# Autodesk Inventor assembly: EnsamblajeDodecaedro_V3
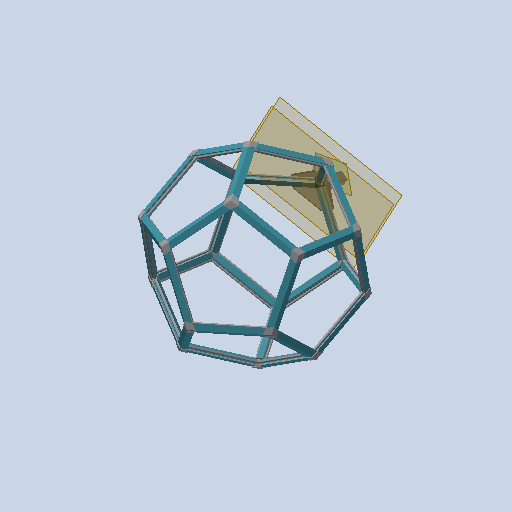
[picture p0: Inventor's stored thumbnail of the model, 512x512]
Saved by Autodesk Inventor 2024 (Build 280153000, 153)
## iProperties
Created: 2023-08-17
Part Number: EnsamblajeDodecaedro_V3
Document SubType Name: Assembly
Designer: sergi
Author: sergi
## Documents named in this file (5)
- C:\Users\sergi\OneDrive\Escritorio\Projects\01. Infinity dodecahedron\Inventor\EnsamblajeDodecaedro_V3.iam
- C:\Users\sergi\OneDrive\Escritorio\Projects\01. Infinity dodecahedron\Inventor\Perfil_V3.ipt
- C:\Users\sergi\OneDrive\Escritorio\Projects\01. Infinity dodecahedron\Inventor\Union.ipt
- C:\Users\sergi\OneDrive\Escritorio\Projects\01. Infinity dodecahedron\Inventor\UnionEntrada.ipt
- C:\Users\sergi\OneDrive\Escritorio\Projects\01. Infinity dodecahedron\Inventor\Base.ipt
## Components (51 placed, 4 different names)
1. Perfil_V3:4 — Coincidencia:1, Coincidencia:2, Coincidencia:3, Coincidencia:19, Coincidencia:20, Coincidencia:21, Coincidencia:154, Coincidencia:155
2. Perfil_V3:5 — Coincidencia:4, Coincidencia:5, Coincidencia:6, Coincidencia:10, Coincidencia:11, Coincidencia:12, Coincidencia:156
3. Perfil_V3:16 — Coincidencia:28, Coincidencia:29, Coincidencia:30, Coincidencia:31, Coincidencia:32, Coincidencia:33
4. Perfil_V3:18 — Coincidencia:7, Coincidencia:8, Coincidencia:9, Coincidencia:55, Coincidencia:56, Coincidencia:57
5. Perfil_V3:25 — Coincidencia:13, Coincidencia:14, Coincidencia:15, Coincidencia:37, Coincidencia:38, Coincidencia:39
6. Perfil_V3:26 — Coincidencia:22, Coincidencia:23, Coincidencia:24, Coincidencia:25, Coincidencia:26, Coincidencia:27
7. Perfil_V3:30 — Coincidencia:16, Coincidencia:17, Coincidencia:18
8. Union:5 — Coincidencia:10, Coincidencia:11, Coincidencia:12, Coincidencia:13, Coincidencia:14, Coincidencia:15, Coincidencia:16, Coincidencia:17, Coincidencia:18
9. Union:6 — Coincidencia:19, Coincidencia:20, Coincidencia:21, Coincidencia:22, Coincidencia:23, Coincidencia:24, Coincidencia:64, Coincidencia:65, Coincidencia:66
10. UnionEntrada:1 — Coincidencia:1, Coincidencia:2, Coincidencia:3, Coincidencia:4, Coincidencia:5, Coincidencia:6, Coincidencia:7, Coincidencia:8, Coincidencia:9
11. Union:7 — Coincidencia:25, Coincidencia:26, Coincidencia:27, Coincidencia:28, Coincidencia:29, Coincidencia:30, Coincidencia:73, Coincidencia:74, Coincidencia:75
12. Union:8 — Coincidencia:31, Coincidencia:32, Coincidencia:33, Coincidencia:34, Coincidencia:35, Coincidencia:36
13. Union:9 — Coincidencia:37, Coincidencia:38, Coincidencia:39, Coincidencia:46, Coincidencia:47, Coincidencia:48, Coincidencia:76, Coincidencia:77, Coincidencia:78
14. Perfil_V3:31 — Coincidencia:34, Coincidencia:35, Coincidencia:36, Coincidencia:79, Coincidencia:80, Coincidencia:81
15. Perfil_V3:32 — Coincidencia:124, Coincidencia:125, Coincidencia:126
16. Perfil_V3:33 — Coincidencia:46, Coincidencia:47, Coincidencia:48
17. Union:10
18. Perfil_V3:34
19. Perfil_V3:35
20. Union:11 — Coincidencia:55, Coincidencia:56, Coincidencia:57
21. Perfil_V3:36
22. Perfil_V3:37 — Coincidencia:64, Coincidencia:65, Coincidencia:66
23. Union:12
24. Perfil_V3:38 — Coincidencia:76, Coincidencia:77, Coincidencia:78
25. Perfil_V3:39 — Coincidencia:73, Coincidencia:74, Coincidencia:75, Coincidencia:106, Coincidencia:107, Coincidencia:114
26. Union:13 — Coincidencia:121, Coincidencia:122, Coincidencia:123
27. Perfil_V3:40
28. Union:14 — Coincidencia:79, Coincidencia:80, Coincidencia:81
29. Perfil_V3:41
30. Perfil_V3:42 — Coincidencia:143
31. Union:15 — Coincidencia:106, Coincidencia:107, Coincidencia:114
32. Union:17 — Coincidencia:148, Coincidencia:149, Coincidencia:150
33. Perfil_V3:44
34. Union:18
35. Perfil_V3:45 — Coincidencia:111, Coincidencia:112, Coincidencia:113
36. Union:19 — Coincidencia:111, Coincidencia:112, Coincidencia:113
37. Perfil_V3:46 — Coincidencia:142, Coincidencia:144
38. Perfil_V3:47 — Coincidencia:121, Coincidencia:122, Coincidencia:123
39. Union:20 — Coincidencia:151, Coincidencia:152, Coincidencia:153
40. Perfil_V3:48
41. Union:21 — Coincidencia:124, Coincidencia:125, Coincidencia:126, Coincidencia:133, Coincidencia:134, Coincidencia:135
42. Perfil_V3:49 — Coincidencia:133, Coincidencia:134, Coincidencia:135
43. Union:22 — Coincidencia:139, Coincidencia:140, Coincidencia:141
44. Perfil_V3:50
45. Union:23 — Coincidencia:142, Coincidencia:143, Coincidencia:144, Coincidencia:145, Coincidencia:146, Coincidencia:147
46. Union:24
47. Perfil_V3:51 — Coincidencia:139, Coincidencia:140, Coincidencia:141
48. Perfil_V3:52 — Coincidencia:145, Coincidencia:146, Coincidencia:147
49. Perfil_V3:53 — Coincidencia:148, Coincidencia:149, Coincidencia:150
50. Perfil_V3:54 — Coincidencia:151, Coincidencia:152, Coincidencia:153
51. Base:1 — Coincidencia:154, Coincidencia:155, Coincidencia:156
## Relationships (150: Mate 150)
- Coincidencia:1 [Mate]: Perfil_V3:4 ↔ UnionEntrada:1
- Coincidencia:2 [Mate]: Perfil_V3:4 ↔ UnionEntrada:1
- Coincidencia:3 [Mate]: Perfil_V3:4 ↔ UnionEntrada:1
- Coincidencia:4 [Mate]: Perfil_V3:5 ↔ UnionEntrada:1
- Coincidencia:5 [Mate]: Perfil_V3:5 ↔ UnionEntrada:1
- Coincidencia:6 [Mate]: Perfil_V3:5 ↔ UnionEntrada:1
- Coincidencia:7 [Mate]: Perfil_V3:18 ↔ UnionEntrada:1
- Coincidencia:8 [Mate]: Perfil_V3:18 ↔ UnionEntrada:1
- Coincidencia:9 [Mate]: Perfil_V3:18 ↔ UnionEntrada:1
- Coincidencia:10 [Mate]: Perfil_V3:5 ↔ Union:5
- Coincidencia:11 [Mate]: Perfil_V3:5 ↔ Union:5
- Coincidencia:12 [Mate]: Perfil_V3:5 ↔ Union:5
- Coincidencia:13 [Mate]: Perfil_V3:25 ↔ Union:5
- Coincidencia:14 [Mate]: Perfil_V3:25 ↔ Union:5
- Coincidencia:15 [Mate]: Perfil_V3:25 ↔ Union:5
- Coincidencia:16 [Mate]: Perfil_V3:30 ↔ Union:5
- Coincidencia:17 [Mate]: Perfil_V3:30 ↔ Union:5
- Coincidencia:18 [Mate]: Perfil_V3:30 ↔ Union:5
- Coincidencia:19 [Mate]: Perfil_V3:4 ↔ Union:6
- Coincidencia:20 [Mate]: Perfil_V3:4 ↔ Union:6
- Coincidencia:21 [Mate]: Perfil_V3:4 ↔ Union:6
- Coincidencia:22 [Mate]: Perfil_V3:26 ↔ Union:6
- Coincidencia:23 [Mate]: Perfil_V3:26 ↔ Union:6
- Coincidencia:24 [Mate]: Perfil_V3:26 ↔ Union:6
- Coincidencia:25 [Mate]: Perfil_V3:26 ↔ Union:7
- Coincidencia:26 [Mate]: Perfil_V3:26 ↔ Union:7
- Coincidencia:27 [Mate]: Perfil_V3:26 ↔ Union:7
- Coincidencia:28 [Mate]: Perfil_V3:16 ↔ Union:7
- Coincidencia:29 [Mate]: Perfil_V3:16 ↔ Union:7
- Coincidencia:30 [Mate]: Perfil_V3:16 ↔ Union:7
- Coincidencia:31 [Mate]: Perfil_V3:16 ↔ Union:8
- Coincidencia:32 [Mate]: Perfil_V3:16 ↔ Union:8
- Coincidencia:33 [Mate]: Perfil_V3:16 ↔ Union:8
- Coincidencia:34 [Mate]: Union:8 ↔ Perfil_V3:31
- Coincidencia:35 [Mate]: Union:8 ↔ Perfil_V3:31
- Coincidencia:36 [Mate]: Union:8 ↔ Perfil_V3:31
- Coincidencia:37 [Mate]: Perfil_V3:25 ↔ Union:9
- Coincidencia:38 [Mate]: Perfil_V3:25 ↔ Union:9
- Coincidencia:39 [Mate]: Perfil_V3:25 ↔ Union:9
- [Mate]: Perfil_V3:32 ↔ Union:10
- [Mate]: Perfil_V3:32 ↔ Union:10
- [Mate]: Perfil_V3:32 ↔ Union:10
- [Mate]: Perfil_V3:33 ↔ Union:10
- [Mate]: Perfil_V3:33 ↔ Union:10
- [Mate]: Perfil_V3:33 ↔ Union:10
- Coincidencia:46 [Mate]: Union:9 ↔ Perfil_V3:33
- Coincidencia:47 [Mate]: Union:9 ↔ Perfil_V3:33
- Coincidencia:48 [Mate]: Union:9 ↔ Perfil_V3:33
- [Mate]: Perfil_V3:34 ↔ Union:11
- [Mate]: Perfil_V3:34 ↔ Union:11
- [Mate]: Perfil_V3:34 ↔ Union:11
- [Mate]: Perfil_V3:35 ↔ Union:11
- [Mate]: Perfil_V3:35 ↔ Union:11
- [Mate]: Perfil_V3:35 ↔ Union:11
- Coincidencia:55 [Mate]: Perfil_V3:18 ↔ Union:11
- Coincidencia:56 [Mate]: Perfil_V3:18 ↔ Union:11
- Coincidencia:57 [Mate]: Perfil_V3:18 ↔ Union:11
- [Mate]: Perfil_V3:36 ↔ Union:12
- [Mate]: Perfil_V3:36 ↔ Union:12
- [Mate]: Perfil_V3:36 ↔ Union:12
- [Mate]: Perfil_V3:37 ↔ Union:12
- [Mate]: Perfil_V3:37 ↔ Union:12
- [Mate]: Perfil_V3:37 ↔ Union:12
- Coincidencia:64 [Mate]: Union:6 ↔ Perfil_V3:37
- Coincidencia:65 [Mate]: Union:6 ↔ Perfil_V3:37
- Coincidencia:66 [Mate]: Union:6 ↔ Perfil_V3:37
- [Mate]: Perfil_V3:38 ↔ Union:13
- [Mate]: Perfil_V3:38 ↔ Union:13
- [Mate]: Perfil_V3:38 ↔ Union:13
- [Mate]: Union:13 ↔ Perfil_V3:40
- [Mate]: Union:13 ↔ Perfil_V3:40
- [Mate]: Union:13 ↔ Perfil_V3:40
- Coincidencia:73 [Mate]: Union:7 ↔ Perfil_V3:39
- Coincidencia:74 [Mate]: Union:7 ↔ Perfil_V3:39
- Coincidencia:75 [Mate]: Union:7 ↔ Perfil_V3:39
- Coincidencia:76 [Mate]: Union:9 ↔ Perfil_V3:38
- Coincidencia:77 [Mate]: Union:9 ↔ Perfil_V3:38
- Coincidencia:78 [Mate]: Union:9 ↔ Perfil_V3:38
- Coincidencia:79 [Mate]: Perfil_V3:31 ↔ Union:14
- Coincidencia:80 [Mate]: Perfil_V3:31 ↔ Union:14
- Coincidencia:81 [Mate]: Perfil_V3:31 ↔ Union:14
- [Mate]: Perfil_V3:41 ↔ Union:15
- [Mate]: Perfil_V3:41 ↔ Union:15
- [Mate]: Perfil_V3:41 ↔ Union:15
- [Mate]: Perfil_V3:42 ↔ Union:15
- [Mate]: Perfil_V3:42 ↔ Union:15
- [Mate]: Perfil_V3:42 ↔ Union:15
- [Mate]: Perfil_V3:41 ↔ Union:17
- [Mate]: Perfil_V3:41 ↔ Union:17
- [Mate]: Perfil_V3:41 ↔ Union:17
- [Mate]: Perfil_V3:44 ↔ Union:18
- [Mate]: Perfil_V3:44 ↔ Union:18
- [Mate]: Perfil_V3:44 ↔ Union:18
- [Mate]: Union:18 ↔ Perfil_V3:45
- [Mate]: Union:18 ↔ Perfil_V3:45
- [Mate]: Union:18 ↔ Perfil_V3:45
- [Mate]: Union:17 ↔ Perfil_V3:44
- [Mate]: Union:17 ↔ Perfil_V3:44
- [Mate]: Union:17 ↔ Perfil_V3:44
- Coincidencia:106 [Mate]: Perfil_V3:39 ↔ Union:15
- Coincidencia:107 [Mate]: Perfil_V3:39 ↔ Union:15
- [Mate]: Union:19 ↔ Perfil_V3:46
- [Mate]: Union:19 ↔ Perfil_V3:46
- [Mate]: Union:19 ↔ Perfil_V3:46
- Coincidencia:111 [Mate]: Perfil_V3:45 ↔ Union:19
- Coincidencia:112 [Mate]: Perfil_V3:45 ↔ Union:19
- Coincidencia:113 [Mate]: Perfil_V3:45 ↔ Union:19
- Coincidencia:114 [Mate]: Perfil_V3:39 ↔ Union:15
- [Mate]: Perfil_V3:47 ↔ Union:20
- [Mate]: Perfil_V3:47 ↔ Union:20
- [Mate]: Perfil_V3:47 ↔ Union:20
- [Mate]: Union:20 ↔ Perfil_V3:48
- [Mate]: Union:20 ↔ Perfil_V3:48
- [Mate]: Union:20 ↔ Perfil_V3:48
- Coincidencia:121 [Mate]: Union:13 ↔ Perfil_V3:47
- Coincidencia:122 [Mate]: Union:13 ↔ Perfil_V3:47
- Coincidencia:123 [Mate]: Union:13 ↔ Perfil_V3:47
- Coincidencia:124 [Mate]: Perfil_V3:32 ↔ Union:21
- Coincidencia:125 [Mate]: Perfil_V3:32 ↔ Union:21
- Coincidencia:126 [Mate]: Perfil_V3:32 ↔ Union:21
- [Mate]: Perfil_V3:49 ↔ Union:22
- [Mate]: Perfil_V3:49 ↔ Union:22
- [Mate]: Perfil_V3:49 ↔ Union:22
- [Mate]: Union:22 ↔ Perfil_V3:50
- [Mate]: Union:22 ↔ Perfil_V3:50
- [Mate]: Union:22 ↔ Perfil_V3:50
- Coincidencia:133 [Mate]: Union:21 ↔ Perfil_V3:49
- Coincidencia:134 [Mate]: Union:21 ↔ Perfil_V3:49
- Coincidencia:135 [Mate]: Union:21 ↔ Perfil_V3:49
- [Mate]: Union:24 ↔ Perfil_V3:51
- [Mate]: Union:24 ↔ Perfil_V3:51
- [Mate]: Union:24 ↔ Perfil_V3:51
- Coincidencia:139 [Mate]: Union:22 ↔ Perfil_V3:51
- Coincidencia:140 [Mate]: Union:22 ↔ Perfil_V3:51
- Coincidencia:141 [Mate]: Union:22 ↔ Perfil_V3:51
- Coincidencia:142 [Mate]: Perfil_V3:46 ↔ Union:23
- Coincidencia:143 [Mate]: Perfil_V3:42 ↔ Union:23
- Coincidencia:144 [Mate]: Perfil_V3:46 ↔ Union:23
- Coincidencia:145 [Mate]: Union:23 ↔ Perfil_V3:52
- Coincidencia:146 [Mate]: Union:23 ↔ Perfil_V3:52
- Coincidencia:147 [Mate]: Union:23 ↔ Perfil_V3:52
- Coincidencia:148 [Mate]: Union:17 ↔ Perfil_V3:53
- Coincidencia:149 [Mate]: Union:17 ↔ Perfil_V3:53
- Coincidencia:150 [Mate]: Union:17 ↔ Perfil_V3:53
- Coincidencia:151 [Mate]: Union:20 ↔ Perfil_V3:54
- Coincidencia:152 [Mate]: Union:20 ↔ Perfil_V3:54
- Coincidencia:153 [Mate]: Union:20 ↔ Perfil_V3:54
- Coincidencia:154 [Mate]: Perfil_V3:4 ↔ Base:1
- Coincidencia:155 [Mate]: Perfil_V3:4 ↔ Base:1
- Coincidencia:156 [Mate]: Perfil_V3:5 ↔ Base:1
## Named parameters: d168_d147 = 0 mm, d169_d148 = 0 mm, d170_d149 = 0 mm, d171_d150 = 0 mm, d172_d151 = 0 mm, d173_d152 = 0 mm, d177_d147 = 0 mm, d178_d148 = 0 mm, d179_d149 = 0 mm, d180_d150 = 0 mm, d181_d151 = 0 mm, d182_d152 = 0 mm, d186_d147 = 0 mm, d187_d148 = 0 mm, d188_d149 = 0 mm, d189_d150 = 0 mm, d190_d151 = 0 mm, d191_d152 = 0 mm, d195_d159 = 0 mm, d196_d160 = 0 mm, d197_d161 = 0 mm, d198_d162 = 0 mm, d199_d163 = 0 mm, d200_d164 = 0 mm, d213_d165 = 0 mm, d214_d166 = 0 mm, d215_d195_d159 = 0 mm, d216_d196_d160 = 0 mm, d217_d197_d161 = 0 mm, d218_d198_d162 = 0 mm, d219_d199_d163 = 0 mm, d220_d200_d164 = 0 mm, d221_d204 = 0 mm, d222_d205 = 0 mm, d223_d206 = 0 mm, d225_d146 = 0 mm, d226_d167 = 0 mm, d227_d141 = 0 mm, d228_d142 = 0 mm, d229_d143 = 0 mm, d230_d144 = 0 mm, d231_d145 = 0 mm, d236_d218_d198_d162 = 0 mm, d237_d219_d199_d163 = 0 mm, d238_d220_d200_d164 = 0 mm, d243_d195_d159 = 0 mm, d244_d196_d160 = 0 mm, d245_d197_d161 = 0 mm, d246_d198_d162 = 0 mm, d247_d199_d163 = 0 mm, d248_d200_d164 = 0 mm, d255_d195_d159 = 0 mm, d256_d196_d160 = 0 mm, d257_d197_d161 = 0 mm, d258_d198_d162 = 0 mm, d259_d199_d163 = 0 mm, d260_d200_d164 = 0 mm, d264_d258_d198_d162 = 0 mm, d265_d259_d199_d163 = 0 mm, d266_d260_d200_d164 = 0 mm
